# Autodesk Inventor assembly: assembly_support
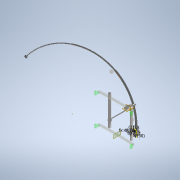
[picture p0: Inventor's stored thumbnail of the model, 180x180]
Saved by Autodesk Inventor 2021 (Build 250183000, 183)
## iProperties
Created: 2021-05-11
Part Number: assembly_support
Document SubType Name: Assembly
Designer: Watchdog
Author: Watchdog
## Documents named in this file (7)
- C:\Users\ocon0143\OneDrive - Flinders\Advn Mech Design Shared\6_Development\2_Design\inventor\support\assembly_support.iam
- C:\Users\ocon0143\OneDrive - Flinders\Advn Mech Design Shared\6_Development\2_Design\inventor\support\roof_bar\ext_roof bar assembly.iam
- C:\Users\ocon0143\OneDrive - Flinders\Advn Mech Design Shared\6_Development\2_Design\inventor\connection\assembly_connector.iam
- C:\Users\ocon0143\OneDrive - Flinders\Advn Mech Design Shared\6_Development\2_Design\inventor\assembly_hoop.iam
- C:\Users\ocon0143\OneDrive - Flinders\Advn Mech Design Shared\6_Development\2_Design\inventor\support\assembly_truss.iam
- C:\Users\ocon0143\OneDrive - Flinders\Advn Mech Design Shared\6_Development\2_Design\inventor\support\support_frame_x.ipt
- C:\Users\ocon0143\OneDrive - Flinders\Advn Mech Design Shared\6_Development\2_Design\inventor\support\support_basePart_truss.ipt
## Components (8 placed, 6 different names)
1. ext_roof bar assembly:1 [sub-assembly] — Flush:6, Flush:7, Flush:8
2. ext_roof bar assembly:2 [sub-assembly] — Flush:3, Flush:4, Flush:5, Flush:6, Flush:7, Flush:8, Flush:9, Mate:11
3. assembly_connector:1 [sub-assembly] — Flush:9, Mate:11, Mate:30
4. assembly_hoop:1 [sub-assembly] — Mate:24, Flush:12, Mate:30
5. assembly_truss:1 [sub-assembly] — Mate:24, Flush:12
6. support_frame_x:1 — Mate:29
7. support_basePart_truss:1 — Mate:29
8. support_basePart_truss:2
## Relationships (12: Flush 8, Mate 4)
- Flush:3: ext_roof bar assembly:2
- Flush:4: ext_roof bar assembly:2
- Flush:5: ext_roof bar assembly:2
- Flush:6 (900 mm): ext_roof bar assembly:1 ↔ ext_roof bar assembly:2
- Flush:7: ext_roof bar assembly:1 ↔ ext_roof bar assembly:2
- Flush:8: ext_roof bar assembly:1 ↔ ext_roof bar assembly:2
- Flush:9: ext_roof bar assembly:2 ↔ assembly_connector:1
- Mate:11: ext_roof bar assembly:2 ↔ assembly_connector:1
- Mate:24: assembly_hoop:1 ↔ assembly_truss:1
- Flush:12: assembly_hoop:1 ↔ assembly_truss:1
- Mate:29: support_frame_x:1 ↔ support_basePart_truss:1
- Mate:30: assembly_connector:1 ↔ assembly_hoop:1
